# Autodesk Inventor assembly: desk_assy
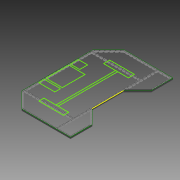
[picture p0: Inventor's stored thumbnail of the model, 180x180]
Saved by Autodesk Inventor 2015 (Build 190159000, 159)
## iProperties
Created: 2017-11-08
Part Number: desk_assy
Document SubType Name: Assembly
Designer: windows7
Author: windows7
## Documents named in this file (3)
- E:\COMPUTER_DESK\desk_assy.iam
- E:\COMPUTER_DESK\desk_clear_top.ipt
- E:\COMPUTER_DESK\top_frame_assy.iam
## Components (2 placed, 2 different names)
1. desk_clear_top:1 — Mate:1, Mate:2
2. top_frame_assy:1 [sub-assembly] — Mate:1, Mate:2
## Relationships (2: Mate 2)
- Mate:1: desk_clear_top:1 ↔ top_frame_assy:1
- Mate:2: desk_clear_top:1 ↔ top_frame_assy:1
